# Autodesk Inventor assembly: McCrea_WALLE
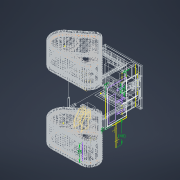
[picture p0: Inventor's stored thumbnail of the model, 180x180]
Saved by Autodesk Inventor 2022 (Build 260153000, 153)
## iProperties
Created: 2022-01-01
Part Number: McCrea_WALLE
Document SubType Name: Assembly
Designer: MatusBarany
Author: MatusBarany
## Documents named in this file (4)
- C:\Users\MatusBarany\Documents\Inventor\wall-e\assembly\McCrea_WALLE.iam
- C:\Users\MatusBarany\Documents\Inventor\wall-e\lukas\McCrea_body_walle.ipt
- C:\Users\MatusBarany\Documents\Inventor\wall-e\matus\right_part.iam
- C:\Users\MatusBarany\Documents\Inventor\wall-e\matus\right_part_MIR.iam
## Components (3 placed, 3 different names)
1. McCrea_body_walle:1 — Flush:1
2. right_part:1 [sub-assembly]
3. right_part_MIR:1 [sub-assembly]
## Relationships (1: Flush 1)
- Flush:1: McCrea_body_walle:1
